# Autodesk Inventor assembly: assembly x
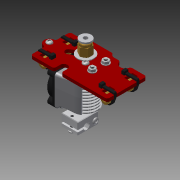
[picture p0: Inventor's stored thumbnail of the model, 180x180]
Saved by Autodesk Inventor 2013 (Build 170138000, 138)
## iProperties
Created: 2015-02-20
Part Number: assembly x
Document SubType Name: Assembly
Designer: Noa Izumi
Author: Noa Izumi
## Documents named in this file (13)
- C:\reprap\TinyBoy_v3_20150220\assembly x.iam
- C:\reprap\TinyBoy_v3_20150220\plastic_part_21.ipt
- C:\reprap\TinyBoy_v3_20150220\plastic_part_13.ipt
- C:\reprap\TinyBoy_v3_20150220\screw_M3_12_hex.ipt
- C:\reprap\TinyBoy_v3_20150220\screw_M3_16_hex.ipt
- C:\reprap\TinyBoy_v3_20150220\washer_M3.ipt
- C:\reprap\TinyBoy_v3_20150220\ring_488.ipt
- C:\reprap\TinyBoy_v3_20150220\nut_M3.ipt
- C:\reprap\TinyBoy_v3_20150220\screw_M3_10_hex.ipt
- C:\reprap\TinyBoy_v3_20150220\fastener_01.ipt
- C:\reprap\TinyBoy_v3_20150220\plastic_part_22.ipt
- C:\reprap\TinyBoy_v3_20150220\e3d_v6.iam
- C:\reprap\TinyBoy_v3_20150220\bearing_603zz.ipt
## Components (27 placed, 12 different names)
1. plastic_part_21:1 — 插入:1, 插入:2, 插入:3, 插入:12, 插入:13, 貼合:1, 貼合:2, 貼合:3, 貼合:4, 相切:1, 相切:2, 相切:3, 相切:4, 相切:5, 相切:6, 相切:7, 相切:8, 插入:16, 插入:17, 角度:1, 角度:2, 角度:3, 角度:4, 插入:22, 插入:23, 角度:5
2. plastic_part_13:1 — 插入:2, 插入:3, 插入:4, 插入:5
3. screw_M3_12_hex:1 — 插入:1
4. screw_M3_16_hex:1 — 插入:10
5. screw_M3_16_hex:2 — 插入:11
6. bearing_603zz:1 — 插入:8, 插入:11
7. bearing_603zz:2 — 插入:9, 插入:10
8. washer_M3:1 — 插入:13, 插入:14
9. washer_M3:2 — 插入:6, 插入:8
10. washer_M3:3 — 插入:5, 插入:7
11. washer_M3:4 — 插入:4, 插入:6
12. washer_M3:5 — 插入:7, 插入:9
13. washer_M3:6 — 插入:12, 插入:15
14. ring_488:1 — 貼合:3, 相切:4, 相切:6, 插入:19
15. ring_488:2 — 貼合:4, 相切:3, 相切:8, 插入:21
16. ring_488:3 — 貼合:1, 相切:1, 相切:5, 插入:18
17. ring_488:4 — 貼合:2, 相切:2, 相切:7, 插入:20
18. nut_M3:1 — 插入:15
19. nut_M3:2 — 插入:14
20. screw_M3_10_hex:1 — 插入:17
21. screw_M3_10_hex:2 — 插入:16
22. fastener_01:1 — 插入:19, 角度:2
23. fastener_01:2 — 插入:20, 角度:3
24. fastener_01:3 — 插入:18, 角度:1
25. fastener_01:4 — 插入:21, 角度:4
26. plastic_part_22:1 — 插入:22, 插入:23, 插入:24
27. e3d_v6:1 [sub-assembly] — 插入:24, 角度:5
## Relationships (41: Insert 24, Tangent 8, Angle 5, Mate 4)
- 插入:1 [Insert]: plastic_part_21:1 ↔ screw_M3_12_hex:1
- 插入:2 [Insert]: plastic_part_21:1 ↔ plastic_part_13:1
- 插入:3 [Insert]: plastic_part_21:1 ↔ plastic_part_13:1
- 插入:4 [Insert]: plastic_part_13:1 ↔ washer_M3:4
- 插入:5 [Insert]: plastic_part_13:1 ↔ washer_M3:3
- 插入:6 [Insert]: washer_M3:2 ↔ washer_M3:4
- 插入:7 [Insert]: washer_M3:3 ↔ washer_M3:5
- 插入:8 [Insert]: bearing_603zz:1 ↔ washer_M3:2
- 插入:9 [Insert]: bearing_603zz:2 ↔ washer_M3:5
- 插入:10 [Insert]: screw_M3_16_hex:1 ↔ bearing_603zz:2
- 插入:11 [Insert]: screw_M3_16_hex:2 ↔ bearing_603zz:1
- 插入:12 [Insert]: plastic_part_21:1 ↔ washer_M3:6
- 插入:13 [Insert]: plastic_part_21:1 ↔ washer_M3:1
- 插入:14 [Insert]: washer_M3:1 ↔ nut_M3:2
- 插入:15 [Insert]: washer_M3:6 ↔ nut_M3:1
- 貼合:1 [Mate]: plastic_part_21:1 ↔ ring_488:3
- 貼合:2 [Mate]: plastic_part_21:1 ↔ ring_488:4
- 貼合:3 [Mate]: plastic_part_21:1 ↔ ring_488:1
- 貼合:4 [Mate]: plastic_part_21:1 ↔ ring_488:2
- 相切:1 [Tangent]: plastic_part_21:1 ↔ ring_488:3
- 相切:2 [Tangent]: plastic_part_21:1 ↔ ring_488:4
- 相切:3 [Tangent]: plastic_part_21:1 ↔ ring_488:2
- 相切:4 [Tangent]: plastic_part_21:1 ↔ ring_488:1
- 相切:5 [Tangent]: plastic_part_21:1 ↔ ring_488:3
- 相切:6 [Tangent]: plastic_part_21:1 ↔ ring_488:1
- 相切:7 [Tangent]: plastic_part_21:1 ↔ ring_488:4
- 相切:8 [Tangent]: plastic_part_21:1 ↔ ring_488:2
- 插入:16 [Insert]: plastic_part_21:1 ↔ screw_M3_10_hex:2
- 插入:17 [Insert]: plastic_part_21:1 ↔ screw_M3_10_hex:1
- 插入:18 [Insert] (2.75 mm): ring_488:3 ↔ fastener_01:3
- 插入:19 [Insert] (2.75 mm): ring_488:1 ↔ fastener_01:1
- 插入:20 [Insert] (2.75 mm): ring_488:4 ↔ fastener_01:2
- 插入:21 [Insert] (2.75 mm): ring_488:2 ↔ fastener_01:4
- 角度:1 [Angle] (0 deg): plastic_part_21:1 ↔ fastener_01:3
- 角度:2 [Angle] (0 deg): plastic_part_21:1 ↔ fastener_01:1
- 角度:3 [Angle] (0 deg): plastic_part_21:1 ↔ fastener_01:2
- 角度:4 [Angle] (0 deg): plastic_part_21:1 ↔ fastener_01:4
- 插入:22 [Insert]: plastic_part_21:1 ↔ plastic_part_22:1
- 插入:23 [Insert]: plastic_part_21:1 ↔ plastic_part_22:1
- 插入:24 [Insert]: plastic_part_22:1 ↔ e3d_v6:1
- 角度:5 [Angle] (0 deg): plastic_part_21:1 ↔ e3d_v6:1
